# Autodesk Inventor assembly: Assembly8.0
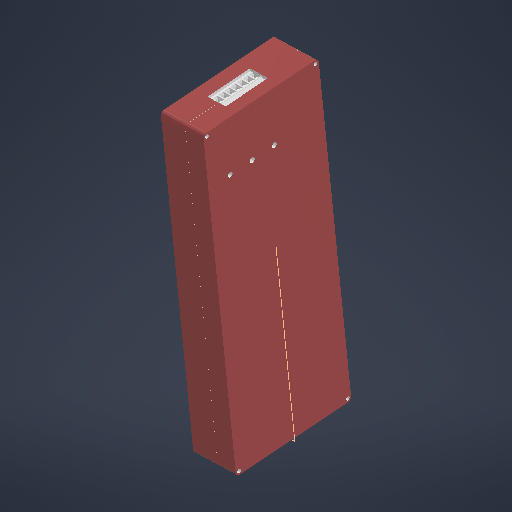
[picture p0: Inventor's stored thumbnail of the model, 512x512]
Saved by Autodesk Inventor 2027 (Build 310192000, 192)
## iProperties
Created: 2026-05-11
Part Number: Assembly8.0
Document SubType Name: Assembly
Designer: giese
Author: giese
## Documents named in this file (6)
- C:\Users\giese\OneDrive\Documents\GitHub\Biphasic-data-acquisition-system\DAQ_design\Assisi\v0.2.1\CAD\Assembly8.0.iam
- C:\Users\giese\OneDrive\Documents\Work\cdaq\cdaq.ipt
- C:\Users\giese\OneDrive\Documents\GitHub\Biphasic-data-acquisition-system\DAQ_design\Assisi\v0.2.1\CAD\cDAQ_Chassis_LowPolyPlaceholder.ipt
- C:\Users\giese\OneDrive\Documents\GitHub\Biphasic-data-acquisition-system\DAQ_design\Assisi\v0.2.1\EDA\assisi_v0.2.1_NEW\assisi_v0.2.1_NEW.ipt
- C:\Users\giese\OneDrive\Documents\GitHub\Biphasic-data-acquisition-system\DAQ_design\Assisi\v0.2.1\CAD\cDAQ_Bottom_Box3.ipt
- C:\Users\giese\OneDrive\Documents\GitHub\Biphasic-data-acquisition-system\DAQ_design\Assisi\v0.2.1\CAD\cDAQ_Lid_Box.ipt
## Components (5 placed, 5 different names)
1. cdaq:1 — Mate:3, Mate:4, Mate:5, Mate:11, Mate:12, Mate:13
2. cDAQ_Chassis_LowPolyPlaceholder:1 — Mate:3, Mate:4, Mate:5, Mate:14, Mate:15, Mate:16, Mate:17
3. assisi_v0.2.1_NEW:1 — Mate:11, Mate:12, Mate:13, Mate:18, Mate:19
4. cDAQ_Bottom_Box3:1 — Mate:14, Mate:15, Mate:16, Mate:17, Mate:18, Mate:19, Mate:20, Flush:1, Flush:2, Mate:21
5. cDAQ_Lid_Box:1 — Mate:20, Flush:1, Flush:2, Mate:21
## Relationships (16: Mate 14, Flush 2)
- Mate:3: cdaq:1 ↔ cDAQ_Chassis_LowPolyPlaceholder:1
- Mate:4: cdaq:1 ↔ cDAQ_Chassis_LowPolyPlaceholder:1
- Mate:5: cdaq:1 ↔ cDAQ_Chassis_LowPolyPlaceholder:1
- Mate:11: cdaq:1 ↔ assisi_v0.2.1_NEW:1
- Mate:12: cdaq:1 ↔ assisi_v0.2.1_NEW:1
- Mate:13: cdaq:1 ↔ assisi_v0.2.1_NEW:1
- Mate:14: cDAQ_Chassis_LowPolyPlaceholder:1 ↔ cDAQ_Bottom_Box3:1
- Mate:15: cDAQ_Chassis_LowPolyPlaceholder:1 ↔ cDAQ_Bottom_Box3:1
- Mate:16: cDAQ_Chassis_LowPolyPlaceholder:1 ↔ cDAQ_Bottom_Box3:1
- Mate:17: cDAQ_Chassis_LowPolyPlaceholder:1 ↔ cDAQ_Bottom_Box3:1
- Mate:18: assisi_v0.2.1_NEW:1 ↔ cDAQ_Bottom_Box3:1
- Mate:19: assisi_v0.2.1_NEW:1 ↔ cDAQ_Bottom_Box3:1
- Mate:20: cDAQ_Bottom_Box3:1 ↔ cDAQ_Lid_Box:1
- Flush:1: cDAQ_Bottom_Box3:1 ↔ cDAQ_Lid_Box:1
- Flush:2: cDAQ_Bottom_Box3:1 ↔ cDAQ_Lid_Box:1
- Mate:21: cDAQ_Bottom_Box3:1 ↔ cDAQ_Lid_Box:1
